# Autodesk Inventor assembly: Spoolholder
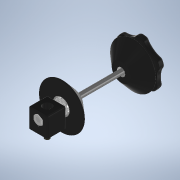
[picture p0: Inventor's stored thumbnail of the model, 180x180]
Saved by Autodesk Inventor 2020.2 (Build 242310000, 310)
## iProperties
Created: 2020-08-25
Part Number: Spoolholder
Document SubType Name: Assembly
Designer: JK
Author: JK
## Documents named in this file (8)
- C:\Users\JK\Documents\Inventor\Anet Upgrade\Spoolholder.iam
- C:\Users\JK\Documents\Inventor\Anet Upgrade\threadedrod.ipt
- C:\Users\JK\Documents\Inventor\Anet Upgrade\Cono 1.ipt
- C:\Users\JK\Documents\Inventor\Anet Upgrade\Bloqueo.ipt
- C:\Users\JK\Documents\Inventor\Anet Upgrade\Bearing608z.ipt
- C:\Users\JK\Documents\Inventor\Anet Upgrade\M8Nut.ipt
- C:\Users\JK\Documents\Inventor\Anet Upgrade\Spoolsupport.ipt
- C:\Users\JK\Documents\Inventor\Anet Upgrade\M8x16socketheadbolt.ipt
## Components (11 placed, 7 different names)
1. threadedrod:1 — Mate:1, Mate:2, Mate:3, Mate:8, Mate:10, Mate:12, Mate:14, Flush:1
2. Cono 1:1 — Mate:2, Mate:4, Mate:6
3. Cono 1:2 — Mate:1, Mate:5, Mate:7
4. Bloqueo:1 — Mate:3, Angle:1, Mate:9
5. Bearing608z:1 — Mate:4, Mate:6, Mate:16
6. Bearing608z:2 — Mate:5, Mate:7, Mate:17
7. M8Nut:1 — Mate:8, Angle:1, Mate:9, Mate:17
8. Spoolsupport:1 — Mate:10, Mate:11, Angle:2, Mate:13, Mate:15, Angle:3, Mate:18, Mate:19, Flush:1
9. M8Nut:2 — Mate:12, Angle:2, Mate:13
10. M8Nut:3 — Mate:14, Mate:15, Angle:3, Mate:16
11. M8x16socketheadbolt:1 — Mate:18, Mate:19
## Relationships (23: Mate 19, Angle 3, Flush 1)
- Mate:1: threadedrod:1 ↔ Cono 1:2
- Mate:2: threadedrod:1 ↔ Cono 1:1
- Mate:3: threadedrod:1 ↔ Bloqueo:1
- Mate:4: Cono 1:1 ↔ Bearing608z:1
- Mate:5: Cono 1:2 ↔ Bearing608z:2
- Mate:6: Cono 1:1 ↔ Bearing608z:1
- Mate:7: Cono 1:2 ↔ Bearing608z:2
- Mate:8: threadedrod:1 ↔ M8Nut:1
- Angle:1 (0 deg): Bloqueo:1 ↔ M8Nut:1
- Mate:9: Bloqueo:1 ↔ M8Nut:1
- Mate:10: threadedrod:1 ↔ Spoolsupport:1
- Mate:11: Spoolsupport:1
- Mate:12: threadedrod:1 ↔ M8Nut:2
- Angle:2 (0 deg): Spoolsupport:1 ↔ M8Nut:2
- Mate:13: Spoolsupport:1 ↔ M8Nut:2
- Mate:14: threadedrod:1 ↔ M8Nut:3
- Mate:15: Spoolsupport:1 ↔ M8Nut:3
- Angle:3 (0 deg): Spoolsupport:1 ↔ M8Nut:3
- Mate:16: Bearing608z:1 ↔ M8Nut:3
- Mate:17: Bearing608z:2 ↔ M8Nut:1
- Mate:18: Spoolsupport:1 ↔ M8x16socketheadbolt:1
- Mate:19: Spoolsupport:1 ↔ M8x16socketheadbolt:1
- Flush:1: threadedrod:1 ↔ Spoolsupport:1
